# Autodesk Inventor assembly: 回転軸フレーム
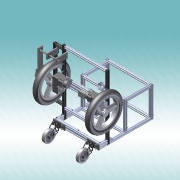
[picture p0: Inventor's stored thumbnail of the model, 180x180]
Saved by Autodesk Inventor 2015 (Build 190159000, 159)
## iProperties
Created: 2016-02-29
Part Number: 回転軸フレーム
Document SubType Name: Assembly
Designer: buzztaka
Author: buzztaka
## Documents named in this file (48)
- C:\Users\buzztaka\Downloads\2kk\回転軸フレーム.iam
- C:\Users\buzztaka\Downloads\2kk\wheel_12inch.ipt
- C:\Users\buzztaka\Downloads\2kk\motor shaft.ipt
- C:\Users\buzztaka\Downloads\2kk\machine key L1.ipt
- C:\Users\buzztaka\Downloads\2kk\machine key L2.ipt
- C:\Users\buzztaka\Downloads\2kk\motor part2.ipt
- C:\Users\buzztaka\Downloads\2kk\wheel-cap.ipt
- C:\Users\buzztaka\Downloads\2kk\kw\wheel-hub.ipt
- C:\Users\buzztaka\Downloads\2kk\caster.ipt
- C:\Users\buzztaka\Downloads\2kk\motor fix plate.ipt
- C:\Users\buzztaka\Downloads\2kk\spacer for caster.ipt
- C:\Users\buzztaka\Downloads\2kk\motor part1.ipt
- C:\Users\buzztaka\Downloads\2kk\Aluminum Extrusions2020-L2.ipt
- C:\Users\buzztaka\Downloads\2kk\Aluminum Extrusions2040-L2.ipt
- C:\Users\buzztaka\Downloads\2kk\Aluminum Extrusions2060-L2.ipt
- C:\Users\buzztaka\Downloads\2kk\Aluminum Extrusions2040-L3.ipt
- C:\Users\buzztaka\Downloads\2kk\Aluminum Extrusions2020-L4.ipt
- C:\Users\buzztaka\Downloads\2kk\Aluminum Extrusions2020-L5.ipt
- C:\Users\buzztaka\Downloads\2kk\Aluminum Extrusions2020-L6.ipt
- C:\Users\buzztaka\Downloads\2kk\Aluminum Extrusions2020-L7.ipt
- C:\Users\buzztaka\Downloads\2kk\hblfsn5.ipt
- C:\Users\buzztaka\Downloads\2kk\hblfsnf5.ipt
- C:\Users\buzztaka\Downloads\2kk\HBLFSSW5.ipt
- C:\Users\buzztaka\Downloads\2kk\hntaj5_5.ipt
- C:\Users\buzztaka\Downloads\2kk\Nat for Aluminum flame.ipt
- C:\Users\buzztaka\Downloads\2kk\Blind Joint Parts - Screw Joints.ipt
- C:\Users\buzztaka\Downloads\2kk\MTi-30.ipt
- C:\Users\buzztaka\Downloads\2kk\M5 washer.ipt
- C:\Users\buzztaka\Downloads\2kk\CapboltM5-10.ipt
- C:\Users\buzztaka\Downloads\2kk\CapboltM5-8.ipt
- C:\Users\buzztaka\Downloads\2kk\spring washer M5.ipt
- C:\Users\buzztaka\Downloads\2kk\spring washer M3.ipt
- C:\Users\buzztaka\Downloads\2kk\Capbolt-M3-6.ipt
- C:\Users\buzztaka\Downloads\2kk\CapboltM5-60.ipt
- C:\Users\buzztaka\Downloads\2kk\CapboltM6-10.ipt
- C:\Users\buzztaka\Downloads\2kk\M3ネジ16mm.ipt
- C:\Users\buzztaka\Downloads\2kk\washer M5.ipt
- C:\Users\buzztaka\Downloads\2kk\kw\HFSB5-2020-550-LCH-RWV-AH30-BH240-CH280-DH442-EH462.ipt
- C:\Users\buzztaka\Downloads\2kk\kw\HFSB5-2020-55-TPW.ipt
- C:\Users\buzztaka\Downloads\2kk\kw\HFSB5-2020-432-LCH-RCH-AH40-BH65.ipt
- C:\Users\buzztaka\Downloads\2kk\kw\HFSB5-2020-550-LCH-RWV-AH30-BH60-CH85-DH240-EH280-AP442.ipt
- C:\Users\buzztaka\Downloads\2kk\kw\C-SFL6901ZZ.ipt
- C:\Users\buzztaka\Downloads\2kk\回転軸取り付け板.ipt
- C:\Users\buzztaka\Downloads\2kk\回転軸.ipt
- C:\Users\buzztaka\Downloads\2kk\kw\タイヤアーム.ipt
- C:\Users\buzztaka\Downloads\2kk\kw\meh-30-pエンコーダ.ipt
- C:\Users\buzztaka\Downloads\2kk\kw\スプリングフランジ用ワッシャー（座金）.ipt
- C:\Users\buzztaka\Downloads\2kk\kw\スプリングフランジ0.1mm.ipt
## Components (59 placed, 19 different names)
1. wheel_12inch
2. wheel-cap
3. wheel-hub
4. hblfsn5
5. hblfsnf5:1
6. hblfsnf5:2
7. HBLFSSW5
8. hntaj5_5:1
9. hntaj5_5:2
10. hntaj5_5:3
11. hntaj5_5:4
12. hntaj5_5:5
13. hntaj5_5:6
14. hntaj5_5:12
15. hntaj5_5:16
16. hntaj5_5:17
17. hntaj5_5:18
18. hntaj5_5:19
19. hntaj5_5:20
20. hntaj5_5:21
21. hntaj5_5:22
22. hntaj5_5:23
23. hntaj5_5:24
24. hntaj5_5:25
25. wheel_12inch:1
26. wheel-cap:1
27. wheel-hub:1
28. MTi-30
29. hblfsn5:1
30. hblfsnf5:3
31. hntaj5_5:26
32. hntaj5_5:27
33. hntaj5_5:28
34. hntaj5_5:35
35. hntaj5_5:36
36. hntaj5_5:37
37. hntaj5_5:38
38. hntaj5_5:39
39. hntaj5_5:40
40. hntaj5_5:41
41. hntaj5_5:42
42. HFSB5-2020-550-LCH-RWV-AH30-BH240-CH280-DH442-EH462:2 — 挿入:3, 挿入:4
43. HFSB5-2020-55-TPW:1 — 挿入:26, 挿入:29
44. HFSB5-2020-55-TPW:2 — 挿入:27, 挿入:28
45. HFSB5-2020-550-LCH-RWV-AH30-BH60-CH85-DH240-EH280-AP442:1 — 挿入:26, 挿入:27, 挿入:32, 挿入:33
46. HFSB5-2020-432-LCH-RCH-AH40-BH65:1 — 挿入:28, 挿入:29, 挿入:37, 挿入:38
47. C-SFL6901ZZ:2 — 挿入:39
48. 回転軸取り付け板:2 — 挿入:32, 挿入:33
49. C-SFL6901ZZ:3
50. 回転軸取り付け板:3 — 挿入:37, 挿入:38
51. 回転軸:1 — 挿入:39, 挿入:41
52. C-SFL6901ZZ:4 — 挿入:40, 挿入:41
53. タイヤアーム:1 — 挿入:40, 挿入:42, 挿入:48, 挿入:49
54. C-SFL6901ZZ:5 — 挿入:42
55. meh-30-pエンコーダ:1
56. スプリングフランジ用ワッシャー（座金）:1
57. スプリングフランジ用ワッシャー（座金）:2
58. スプリングフランジ用ワッシャー（座金）:3
59. スプリングフランジ0.1mm:1 — 挿入:48, 挿入:49
## Relationships (25: Insert 25)
- 挿入:3 [Insert]: HFSB5-2020-550-LCH-RWV-AH30-BH240-CH280-DH442-EH462:2
- 挿入:4 [Insert]: HFSB5-2020-550-LCH-RWV-AH30-BH240-CH280-DH442-EH462:2
- [Insert]: HFSB5-2020-550-LCH-RWV-AH30-BH60-CH85-DH240-EH280-AP442:1
- [Insert]: HFSB5-2020-550-LCH-RWV-AH30-BH60-CH85-DH240-EH280-AP442:1
- 挿入:26 [Insert]: HFSB5-2020-55-TPW:1 ↔ HFSB5-2020-550-LCH-RWV-AH30-BH60-CH85-DH240-EH280-AP442:1
- 挿入:27 [Insert]: HFSB5-2020-55-TPW:2 ↔ HFSB5-2020-550-LCH-RWV-AH30-BH60-CH85-DH240-EH280-AP442:1
- 挿入:28 [Insert]: HFSB5-2020-55-TPW:2 ↔ HFSB5-2020-432-LCH-RCH-AH40-BH65:1
- 挿入:29 [Insert]: HFSB5-2020-55-TPW:1 ↔ HFSB5-2020-432-LCH-RCH-AH40-BH65:1
- [Insert]: C-SFL6901ZZ:2 ↔ 回転軸取り付け板:2
- 挿入:32 [Insert]: HFSB5-2020-550-LCH-RWV-AH30-BH60-CH85-DH240-EH280-AP442:1 ↔ 回転軸取り付け板:2
- 挿入:33 [Insert]: HFSB5-2020-550-LCH-RWV-AH30-BH60-CH85-DH240-EH280-AP442:1 ↔ 回転軸取り付け板:2
- [Insert]: C-SFL6901ZZ:3 ↔ 回転軸取り付け板:3
- 挿入:37 [Insert]: HFSB5-2020-432-LCH-RCH-AH40-BH65:1 ↔ 回転軸取り付け板:3
- 挿入:38 [Insert]: HFSB5-2020-432-LCH-RCH-AH40-BH65:1 ↔ 回転軸取り付け板:3
- 挿入:39 [Insert] (-20 mm): C-SFL6901ZZ:2 ↔ 回転軸:1
- 挿入:40 [Insert]: C-SFL6901ZZ:4 ↔ タイヤアーム:1
- 挿入:41 [Insert] (-10 mm): 回転軸:1 ↔ C-SFL6901ZZ:4
- 挿入:42 [Insert]: タイヤアーム:1 ↔ C-SFL6901ZZ:5
- [Insert]: meh-30-pエンコーダ:1 ↔ スプリングフランジ用ワッシャー（座金）:2
- [Insert]: meh-30-pエンコーダ:1 ↔ スプリングフランジ用ワッシャー（座金）:1
- [Insert]: meh-30-pエンコーダ:1 ↔ スプリングフランジ用ワッシャー（座金）:3
- [Insert]: スプリングフランジ用ワッシャー（座金）:2 ↔ スプリングフランジ0.1mm:1
- [Insert]: スプリングフランジ用ワッシャー（座金）:3 ↔ スプリングフランジ0.1mm:1
- 挿入:48 [Insert]: タイヤアーム:1 ↔ スプリングフランジ0.1mm:1
- 挿入:49 [Insert]: タイヤアーム:1 ↔ スプリングフランジ0.1mm:1
## Named parameters: d53_d52 = 0 mm, d58_d52 = 0 mm
